# Autodesk Inventor assembly: roller
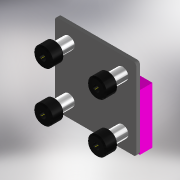
[picture p0: Inventor's stored thumbnail of the model, 180x180]
Saved by Autodesk Inventor 2020 (Build 240168000, 168)
## iProperties
Created: 2020-06-18
Part Number: roller
Document SubType Name: Assembly
Designer: pc-konvi
Author: pc-konvi
## Documents named in this file (5)
- C:\Users\pc-konvi\Documents\Lobola\open_source_scrabble\lobola - rapid prototype\roller.iam
- C:\Users\pc-konvi\Documents\Lobola\open_source_scrabble\lobola - rapid prototype\wheel.ipt
- C:\Users\pc-konvi\Documents\Lobola\open_source_scrabble\lobola - rapid prototype\wheel_plate.ipt
- C:\Users\pc-konvi\Documents\Lobola\open_source_scrabble\lobola - rapid prototype\wheel_spacer.ipt
- C:\Users\pc-konvi\Documents\Lobola\open_source_scrabble\lobola - rapid prototype\roller_support.ipt
## Components (10 placed, 4 different names)
1. wheel_plate:1 — Mate:1, Mate:2, Flush:1, Mate:5, Mate:9, Flush:2, Flush:3
2. roller_support:1 — Mate:9, Flush:2, Flush:3
3. wheel_spacer:1 — Mate:7, Mate:8
4. wheel:1 — Mate:5, Mate:6, Mate:7, Mate:8
5. wheel_spacer:2
6. wheel:2
7. wheel_spacer:3
8. wheel:3
9. wheel_spacer:4
10. wheel:4
## Component patterns: (4 elements, first: wheel_spacer:1 + wheel:1)
## Relationships (10: Mate 7, Flush 3)
- Mate:1: wheel_plate:1
- Mate:2: wheel_plate:1
- Flush:1: wheel_plate:1
- Mate:5 (16 mm): wheel_plate:1 ↔ wheel:1
- Mate:6 (21.5 mm): wheel:1
- Mate:7: wheel_spacer:1 ↔ wheel:1
- Mate:8: wheel_spacer:1 ↔ wheel:1
- Mate:9: wheel_plate:1 ↔ roller_support:1
- Flush:2: wheel_plate:1 ↔ roller_support:1
- Flush:3: wheel_plate:1 ↔ roller_support:1
